# Autodesk Inventor assembly: GE-12072
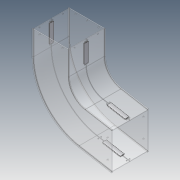
[picture p0: Inventor's stored thumbnail of the model, 180x180]
Saved by Autodesk Inventor 2012 (Build 160160000, 160)
## iProperties
Created: 2011-09-22
Part Number: GE-12072
Document SubType Name: Assembly
Designer: dfoster
Description: Chute 1, Assembly
Title: Chute 1, Assembly
Author: dfoster
## Documents named in this file (4)
- C:\Data Folder\FRC 2012 Field\Components\GE-12072.iam
- C:\Data Folder\FRC 2012 Field\Components\GE-12071.iam
- C:\Data Folder\FRC 2012 Field\Components\GE-12070.iam
- C:\Data Folder\FRC 2012 Field\Components\GE-12072-01.ipt
## Components (6 placed, 3 different names)
1. GE-12071:1 [sub-assembly] — Flush:1, Flush:2, Mate:1, Mate:2, Mate:3, Flush:3, Mate:4, Mate:5, Mate:7, Mate:8, Mate:9, Mate:10
2. GE-12070:1 [sub-assembly] — Flush:1, Flush:2, Mate:1, Mate:6, Mate:11
3. GE-12072-01:1 — Mate:2, Mate:3, Flush:3, Flush:4
4. GE-12072-01:2 — Mate:4, Mate:5, Flush:4
5. GE-12072-01:3 — Mate:6, Mate:7, Mate:8
6. GE-12072-01:4 — Mate:9, Mate:10, Mate:11
## Relationships (15: Mate 11, Flush 4)
- Flush:1: GE-12071:1 ↔ GE-12070:1
- Flush:2: GE-12071:1 ↔ GE-12070:1
- Mate:1 (3.175 mm): GE-12071:1 ↔ GE-12070:1
- Mate:2: GE-12071:1 ↔ GE-12072-01:1
- Mate:3: GE-12071:1 ↔ GE-12072-01:1
- Flush:3 (-19.05 mm): GE-12071:1 ↔ GE-12072-01:1
- Mate:4: GE-12071:1 ↔ GE-12072-01:2
- Mate:5: GE-12071:1 ↔ GE-12072-01:2
- Flush:4: GE-12072-01:1 ↔ GE-12072-01:2
- Mate:6: GE-12070:1 ↔ GE-12072-01:3
- Mate:7: GE-12071:1 ↔ GE-12072-01:3
- Mate:8 (50.8 mm): GE-12071:1 ↔ GE-12072-01:3
- Mate:9: GE-12071:1 ↔ GE-12072-01:4
- Mate:10: GE-12071:1 ↔ GE-12072-01:4
- Mate:11 (19.05 mm): GE-12070:1 ↔ GE-12072-01:4
